# Autodesk Inventor assembly: SUSPENSION UNIT
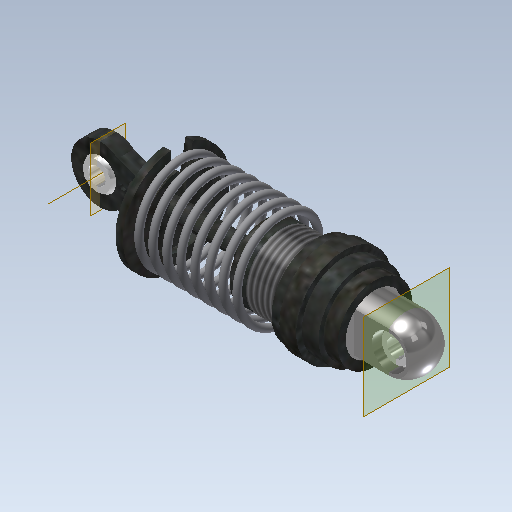
[picture p0: Inventor's stored thumbnail of the model, 512x512]
Saved by Autodesk Inventor 2020 (Build 240168000, 168)
## iProperties
Created: 2015-04-18
Part Number: SUSPENSION UNIT
Document SubType Name: Assembly
Designer: Station9
Author: Station9
## Documents named in this file (10)
- C:\Users\0x6f736f646f\Downloads\rc-car-16.snapshot.3\SUSPENSION UNIT.iam
- C:\Users\0x6f736f646f\Downloads\rc-car-16.snapshot.3\500-102.ipt
- C:\Users\0x6f736f646f\Downloads\rc-car-16.snapshot.3\500-106.ipt
- C:\Users\0x6f736f646f\Downloads\rc-car-16.snapshot.3\500-105.ipt
- C:\Users\0x6f736f646f\Downloads\rc-car-16.snapshot.3\500-109.ipt
- C:\Users\0x6f736f646f\Downloads\rc-car-16.snapshot.3\500-104.ipt
- C:\Users\0x6f736f646f\Downloads\rc-car-16.snapshot.3\500-103.ipt
- C:\Users\0x6f736f646f\Downloads\rc-car-16.snapshot.3\500-100.ipt
- C:\Users\0x6f736f646f\Downloads\rc-car-16.snapshot.3\Compression Spring 16.ipt
- C:\Users\0x6f736f646f\Downloads\rc-car-16.snapshot.3\500-107.ipt
## Components (10 placed, 9 different names)
1. 500-102:1 — Mate:9, Mate:13
2. 500-106:1 — Mate:6, Flush:1, Mate:12, Angle:3, Mate:15
3. 500-105:1 — Insert:1, Mate:3, Mate:4
4. 500-109:1 — Mate:1, Mate:2, Angle:2
5. 500-104:1 — Mate:5, Mate:6, Mate:8, Mate:9, Mate:11, Mate:14
6. 500-103:1 — Mate:1, Mate:2, Insert:1, Mate:5, Angle:2, Mate:11
7. 500-100:1 — Mate:8, Flush:1, Mate:13
8. Compression Spring 16:1 — Mate:3, Mate:4
9. 500-109:2 — Mate:12, Angle:3
10. 500-107:1 — Mate:14, Mate:15
## Relationships (17: Mate 13, Angle 2, Insert 1, Flush 1)
- Mate:1: 500-109:1 ↔ 500-103:1
- Mate:2: 500-109:1 ↔ 500-103:1
- Insert:1: 500-105:1 ↔ 500-103:1
- Mate:3: 500-105:1 ↔ Compression Spring 16:1
- Mate:4: 500-105:1 ↔ Compression Spring 16:1
- Mate:5: 500-104:1 ↔ 500-103:1
- Mate:6: 500-106:1 ↔ 500-104:1
- Mate:8: 500-104:1 ↔ 500-100:1
- Mate:9: 500-102:1 ↔ 500-104:1
- Flush:1: 500-106:1 ↔ 500-100:1
- Angle:2 (0 deg): 500-109:1 ↔ 500-103:1
- Mate:11: 500-104:1 ↔ 500-103:1
- Mate:12: 500-106:1 ↔ 500-109:2
- Angle:3 (0 deg): 500-106:1 ↔ 500-109:2
- Mate:13: 500-102:1 ↔ 500-100:1
- Mate:14: 500-104:1 ↔ 500-107:1
- Mate:15: 500-106:1 ↔ 500-107:1
